# Autodesk Inventor assembly: iPadHolderAssembly
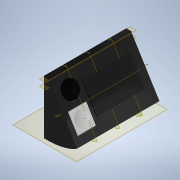
[picture p0: Inventor's stored thumbnail of the model, 180x180]
Saved by Autodesk Inventor 2021.3 (Build 253353000, 353)
## iProperties
Created: 2020-11-06
Part Number: iPadHolderAssembly
Document SubType Name: Assembly
Designer: gisen
Author: gisen
## Documents named in this file (5)
- C:\Users\gisen\GitProjects\CAD-Data\CuboidAccessories\SecurityBox\Assemblies\DisplayHolderAssembly.iam
- C:\Users\gisen\GitProjects\CAD-Data\CuboidAccessories\SecurityBox\3DPrintedParts\DisplayHolder.ipt
- C:\Users\gisen\GitProjects\CAD-Data\Devices\Microphone\Microphone_iGOKU.ipt
- C:\Users\gisen\GitProjects\CAD-Data\Devices\Display\Display_EVICIV7Inch.ipt
- C:\Users\gisen\GitProjects\CAD-Data\Devices\Button\Button.ipt
## Components (4 placed, 4 different names)
1. DisplayHolder:1 — メイト:4, メイト:5, メイト:6, メイト:7, フラッシュ:1, フラッシュ:3, メイト:8, メイト:9, フラッシュ:5, メイト:10, メイト:11, メイト:12
2. Microphone_iGOKU:1 — メイト:7, メイト:9, メイト:10
3. Display_EVICIV7Inch:1 — フラッシュ:1, メイト:8, フラッシュ:5
4. Button:1 — フラッシュ:3, メイト:11, メイト:12
## Relationships (12: Mate 9, Flush 3)
- メイト:4 [Mate]: DisplayHolder:1
- メイト:5 [Mate]: DisplayHolder:1
- メイト:6 [Mate]: DisplayHolder:1
- メイト:7 [Mate] (-5.5 mm): DisplayHolder:1 ↔ Microphone_iGOKU:1
- フラッシュ:1 [Flush] (2 mm): DisplayHolder:1 ↔ Display_EVICIV7Inch:1
- フラッシュ:3 [Flush] (1 mm): DisplayHolder:1 ↔ Button:1
- メイト:8 [Mate]: DisplayHolder:1 ↔ Display_EVICIV7Inch:1
- メイト:9 [Mate] (-50 mm): DisplayHolder:1 ↔ Microphone_iGOKU:1
- フラッシュ:5 [Flush] (30 mm): DisplayHolder:1 ↔ Display_EVICIV7Inch:1
- メイト:10 [Mate] (50 mm): DisplayHolder:1 ↔ Microphone_iGOKU:1
- メイト:11 [Mate] (-50 mm): DisplayHolder:1 ↔ Button:1
- メイト:12 [Mate] (-60 mm): DisplayHolder:1 ↔ Button:1
